# Autodesk Inventor assembly: PLATAFORMA_ASSEMBLY
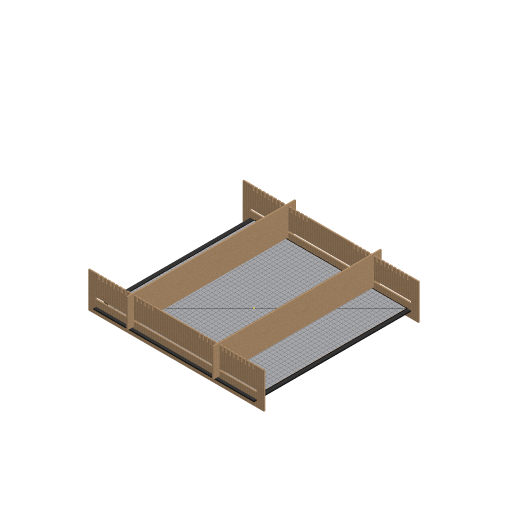
[picture p0: Inventor's stored thumbnail of the model, 512x512]
Saved by Autodesk Inventor 2024.2 (Build 282272000, 272)
## iProperties
Created: 2024-11-02
Part Number: PLATAFORMA_ASSEMBLY
Document SubType Name: Assembly
Designer: jrcer
Author: jrcer
## Documents named in this file (5)
- C:\Users\jrcer\Universidad\S10_2024\TDG\Tesis\Modelos\PLATAFORMA_ASSEMBLY.iam
- C:\Users\jrcer\Universidad\S10_2024\TDG\Tesis\Modelos\42X42_BASE_PLATAFORMA.ipt
- C:\Users\jrcer\Universidad\S10_2024\TDG\Tesis\Modelos\40X40_CUADRICULA_PLATAFORMA.ipt
- C:\Users\jrcer\Universidad\S10_2024\TDG\Tesis\Modelos\PARED_MODULAR.ipt
- C:\Users\jrcer\Universidad\S10_2024\TDG\Tesis\Modelos\PARED_ESTRUCTURAL.ipt
## Components (6 placed, 4 different names)
1. 42X42_BASE_PLATAFORMA:1 — Mate:1, Mate:2, Mate:3, Mate:4, Mate:5, Mate:6, Mate:13, Flush:1, Flush:2
2. PARED_MODULAR:1 — Mate:1, Mate:2, Mate:3, Mate:14
3. PARED_MODULAR:2 — Mate:4, Mate:5, Mate:6, Mate:8, Mate:9, Mate:11, Mate:12, Mate:15
4. PARED_ESTRUCTURAL:1 — Mate:8, Mate:9, Mate:15
5. PARED_ESTRUCTURAL:2 — Mate:11, Mate:12, Mate:14
6. 40X40_CUADRICULA_PLATAFORMA:1 — Mate:13, Flush:1, Flush:2
## Relationships (15: Mate 13, Flush 2)
- Mate:1 (-10 mm): 42X42_BASE_PLATAFORMA:1 ↔ PARED_MODULAR:1
- Mate:2: 42X42_BASE_PLATAFORMA:1 ↔ PARED_MODULAR:1
- Mate:3: 42X42_BASE_PLATAFORMA:1 ↔ PARED_MODULAR:1
- Mate:4 (-10 mm): 42X42_BASE_PLATAFORMA:1 ↔ PARED_MODULAR:2
- Mate:5: 42X42_BASE_PLATAFORMA:1 ↔ PARED_MODULAR:2
- Mate:6: 42X42_BASE_PLATAFORMA:1 ↔ PARED_MODULAR:2
- Mate:8: PARED_MODULAR:2 ↔ PARED_ESTRUCTURAL:1
- Mate:9: PARED_MODULAR:2 ↔ PARED_ESTRUCTURAL:1
- Mate:11: PARED_MODULAR:2 ↔ PARED_ESTRUCTURAL:2
- Mate:12: PARED_MODULAR:2 ↔ PARED_ESTRUCTURAL:2
- Mate:13: 42X42_BASE_PLATAFORMA:1 ↔ 40X40_CUADRICULA_PLATAFORMA:1
- Flush:1 (10 mm): 42X42_BASE_PLATAFORMA:1 ↔ 40X40_CUADRICULA_PLATAFORMA:1
- Flush:2 (10 mm): 42X42_BASE_PLATAFORMA:1 ↔ 40X40_CUADRICULA_PLATAFORMA:1
- Mate:14: PARED_MODULAR:1 ↔ PARED_ESTRUCTURAL:2
- Mate:15: PARED_MODULAR:2 ↔ PARED_ESTRUCTURAL:1
